# Autodesk Inventor assembly: cremalheira pronta
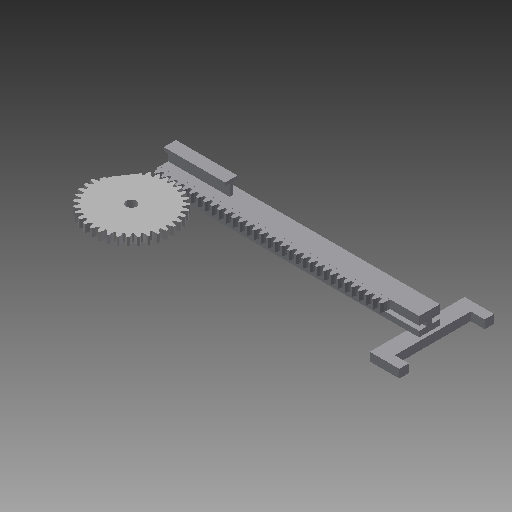
[picture p0: Inventor's stored thumbnail of the model, 512x512]
Saved by Autodesk Inventor 2019 (Build 230136000, 136)
## iProperties
Created: 2018-06-04
Part Number: cremalheira pronta
Material: Genérico
Document SubType Name: Assembly
Designer: Ernandes
Author: Ernandes
## Documents named in this file (4)
- C:\Users\Ernandes\Google Drive (sguimaraaes@gmail.com)\TCC\3D\lançador.inventor\cremalheira pronta.iam
- C:\Users\Ernandes\Google Drive (sguimaraaes@gmail.com)\TCC\3D\lançador.inventor\trilho sem cremalheira.ipt
- C:\Users\Ernandes\Google Drive (sguimaraaes@gmail.com)\TCC\3D\lançador.inventor\cremalheira.ipt
- C:\Users\Ernandes\Google Drive (sguimaraaes@gmail.com)\TCC\3D\lançador.inventor\Engrenagem reta22.ipt
## Components (3 placed, 3 different names)
1. trilho sem cremalheira:1 — Coincidência:1, Coincidência:2
2. cremalheira:1 — Coincidência:1, Coincidência:2
3. Engrenagem reta2:1
## Relationships (2: Mate 2)
- Coincidência:1 [Mate]: trilho sem cremalheira:1 ↔ cremalheira:1
- Coincidência:2 [Mate]: trilho sem cremalheira:1 ↔ cremalheira:1
